# Autodesk Inventor assembly: Shooter Assembly
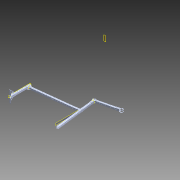
[picture p0: Inventor's stored thumbnail of the model, 180x180]
Saved by Autodesk Inventor 2014 (Build 180170000, 170)
## iProperties
Created: 2014-01-05
Part Number: Shooter Assembly
Document SubType Name: Assembly
Designer: Andrew Toennies
Mass: 581.2 g
Surface Area: 3707.46 cm^2
Volume: 214.465 cm^3
Density: 2.71 g/cm^3
Author: Andrew Toennies
## Documents named in this file (9)
- C:\Users\Andrew Toennies\Documents\GitHub\2014buildCAD\Shooter\Shooter Assembly.iam
- C:\Users\Andrew Toennies\Documents\GitHub\2014buildCAD\Shooter\Vex Pro 1x1 rectangular tubing 12 in length.ipt
- C:\Users\Andrew Toennies\Documents\GitHub\2014buildCAD\Shooter\Vex Pro End Bearing Mount.ipt
- C:\Users\Andrew Toennies\Documents\GitHub\2014buildCAD\Shooter\Vex Pro 1x1 rectangular tubing 27 in length.ipt
- C:\Users\Andrew Toennies\Documents\GitHub\2014buildCAD\Shooter\Vex Pro 1x1 rectangular tubing 24 in length.ipt
- C:\Users\Andrew Toennies\Documents\GitHub\2014buildCAD\Shooter\Vex Pro T gusset.ipt
- C:\Users\Andrew Toennies\Documents\GitHub\2014buildCAD\Shooter\Vex Pro Corner Gusset.ipt
- C:\Users\Andrew Toennies\Documents\GitHub\2014buildCAD\Shooter\Vex Pro 1x1 rectangular tubing 13 in length.ipt
- C:\Users\Andrew Toennies\Documents\GitHub\2014buildCAD\Shooter\Vex Pro Side Bearing Gusset.ipt
## Components (14 placed, 8 different names)
1. Vex Pro 1x1 rectangular tubing 12 in length:1 — Flush:1, Insert:9, Insert:10, Insert:11, Insert:12, Insert:17, Insert:18, Insert:19, Insert:20, Flush:4
2. Vex Pro 1x1 rectangular tubing 27 in length:1 — Flush:1, Insert:5, Insert:6, Insert:7, Insert:8, Flush:2, Mate:2, Mate:5
3. Vex Pro 1x1 rectangular tubing 24 in length:1 — Flush:2, Mate:2, Insert:13, Insert:14, Insert:15, Insert:16, Flush:3, Mate:6
4. Vex Pro T gusset:1 — Insert:5, Insert:6, Mate:6
5. Vex Pro T gusset:2 — Insert:7, Insert:8
6. Vex Pro Corner Gusset:1 — Insert:9, Insert:10, Flush:6
7. Vex Pro Corner Gusset:2 — Insert:11, Insert:12
8. Vex Pro End Bearing Mount:3 — Insert:13, Insert:14
9. Vex Pro End Bearing Mount:4 — Insert:15, Insert:16, Mate:4
10. Vex Pro 1x1 rectangular tubing 13 in length:1 — Mate:4, Flush:3, Insert:21, Insert:22, Insert:23, Insert:24
11. Vex Pro End Bearing Mount:5 — Insert:21, Insert:22
12. Vex Pro End Bearing Mount:6 — Insert:23, Insert:24
13. Vex Pro Side Bearing Gusset:1 — Insert:17, Insert:18
14. Vex Pro Side Bearing Gusset:2 — Insert:19, Insert:20, Mate:5
## Relationships (30: Insert 20, Flush 6, Mate 4)
- Flush:1: Vex Pro 1x1 rectangular tubing 12 in length:1 ↔ Vex Pro 1x1 rectangular tubing 27 in length:1
- Insert:5: Vex Pro 1x1 rectangular tubing 27 in length:1 ↔ Vex Pro T gusset:1
- Insert:6: Vex Pro 1x1 rectangular tubing 27 in length:1 ↔ Vex Pro T gusset:1
- Insert:7: Vex Pro 1x1 rectangular tubing 27 in length:1 ↔ Vex Pro T gusset:2
- Insert:8: Vex Pro 1x1 rectangular tubing 27 in length:1 ↔ Vex Pro T gusset:2
- Flush:2: Vex Pro 1x1 rectangular tubing 27 in length:1 ↔ Vex Pro 1x1 rectangular tubing 24 in length:1
- Mate:2: Vex Pro 1x1 rectangular tubing 27 in length:1 ↔ Vex Pro 1x1 rectangular tubing 24 in length:1
- Insert:9: Vex Pro 1x1 rectangular tubing 12 in length:1 ↔ Vex Pro Corner Gusset:1
- Insert:10: Vex Pro 1x1 rectangular tubing 12 in length:1 ↔ Vex Pro Corner Gusset:1
- Insert:11: Vex Pro 1x1 rectangular tubing 12 in length:1 ↔ Vex Pro Corner Gusset:2
- Insert:12: Vex Pro 1x1 rectangular tubing 12 in length:1 ↔ Vex Pro Corner Gusset:2
- Insert:13: Vex Pro 1x1 rectangular tubing 24 in length:1 ↔ Vex Pro End Bearing Mount:3
- Insert:14: Vex Pro 1x1 rectangular tubing 24 in length:1 ↔ Vex Pro End Bearing Mount:3
- Insert:15: Vex Pro 1x1 rectangular tubing 24 in length:1 ↔ Vex Pro End Bearing Mount:4
- Insert:16: Vex Pro 1x1 rectangular tubing 24 in length:1 ↔ Vex Pro End Bearing Mount:4
- Mate:4: Vex Pro End Bearing Mount:4 ↔ Vex Pro 1x1 rectangular tubing 13 in length:1
- Flush:3: Vex Pro 1x1 rectangular tubing 24 in length:1 ↔ Vex Pro 1x1 rectangular tubing 13 in length:1
- Insert:17: Vex Pro 1x1 rectangular tubing 12 in length:1 ↔ Vex Pro Side Bearing Gusset:1
- Insert:18: Vex Pro 1x1 rectangular tubing 12 in length:1 ↔ Vex Pro Side Bearing Gusset:1
- Insert:19: Vex Pro 1x1 rectangular tubing 12 in length:1 ↔ Vex Pro Side Bearing Gusset:2
- Insert:20: Vex Pro 1x1 rectangular tubing 12 in length:1 ↔ Vex Pro Side Bearing Gusset:2
- Mate:5: Vex Pro 1x1 rectangular tubing 27 in length:1 ↔ Vex Pro Side Bearing Gusset:2
- Flush:4: Vex Pro 1x1 rectangular tubing 12 in length:1
- Mate:6: Vex Pro 1x1 rectangular tubing 24 in length:1 ↔ Vex Pro T gusset:1
- Flush:5 (-711.2 mm)
- Flush:6 (-1422.4 mm): Vex Pro Corner Gusset:1
- Insert:21: Vex Pro 1x1 rectangular tubing 13 in length:1 ↔ Vex Pro End Bearing Mount:5
- Insert:22: Vex Pro 1x1 rectangular tubing 13 in length:1 ↔ Vex Pro End Bearing Mount:5
- Insert:23: Vex Pro 1x1 rectangular tubing 13 in length:1 ↔ Vex Pro End Bearing Mount:6
- Insert:24: Vex Pro 1x1 rectangular tubing 13 in length:1 ↔ Vex Pro End Bearing Mount:6
